# Autodesk Inventor assembly: Full Chassis - Full Assembly
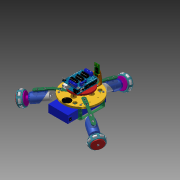
[picture p0: Inventor's stored thumbnail of the model, 180x180]
Saved by Autodesk Inventor 2014 (Build 180170000, 170)
## iProperties
Created: 2014-02-26
Part Number: Full Chassis - Full Assembly
Document SubType Name: Assembly
Designer: Spooner
Author: Spooner
## Documents named in this file (5)
- C:\Users\Spooner\Documents\Inventor\FerretBall Robot\3Pod\Inventor 2014 Files\Full Chassis - Full Assembly.iam
- C:\Users\Spooner\Documents\Inventor\FerretBall Robot\3Pod\Inventor 2014 Files\Main Body - Full Assembly.iam
- C:\Users\Spooner\Documents\Inventor\FerretBall Robot\3Pod\Inventor 2014 Files\Full Motor Arm (1 inch) with Kornylak Wheel.iam
- C:\Users\Spooner\Documents\Inventor\Content Center Files\R2014\en-US\JIS B 1111(1)\JIS B 1111 - M3x10(1).ipt
- C:\Users\Spooner\Documents\Inventor\Content Center Files\R2014\en-US\JIS B 1181 U\JIS B 1181 - B M3.ipt
## Components (16 placed, 4 different names)
1. Main Body - Full Assembly:1 [sub-assembly] — Insert:1, Mate:1, Insert:2, Mate:2, Insert:3, Mate:3, Insert:10, Insert:11, Insert:12, Insert:13, Insert:14, Insert:15
2. Full Motor Arm (1 inch) with Kornylak Wheel:1 [sub-assembly] — Insert:3, Mate:3, Insert:6, Insert:9, Angle:3, Angle:4
3. Full Motor Arm (1 inch) with Kornylak Wheel:2 [sub-assembly] — Insert:2, Mate:2, Insert:7, Insert:8, Angle:1, Angle:2
4. Full Motor Arm (1 inch) with Kornylak Wheel:3 [sub-assembly] — Insert:1, Mate:1, Insert:4, Insert:5, Angle:5, Angle:6
5. JIS B 1111 M3x10:1 — Insert:11
6. JIS B 1111 M3x10:2 — Insert:13
7. JIS B 1111 M3x10:3 — Insert:15
8. JIS B 1111 M3x10:4 — Insert:14
9. JIS B 1111 M3x10:5 — Insert:12
10. JIS B 1111 M3x10:6 — Insert:10
11. JIS B 1181 (unchamfered) - Metric B M3:1 — Insert:4, Angle:6
12. JIS B 1181 (unchamfered) - Metric B M3:2 — Insert:9, Angle:3
13. JIS B 1181 (unchamfered) - Metric B M3:3 — Insert:6, Angle:4
14. JIS B 1181 (unchamfered) - Metric B M3:4 — Insert:7, Angle:2
15. JIS B 1181 (unchamfered) - Metric B M3:5 — Insert:8, Angle:1
16. JIS B 1181 (unchamfered) - Metric B M3:6 — Insert:5, Angle:5
## Relationships (24: Insert 15, Angle 6, Mate 3)
- Insert:1: Main Body - Full Assembly:1 ↔ Full Motor Arm (1 inch) with Kornylak Wheel:3
- Mate:1: Main Body - Full Assembly:1 ↔ Full Motor Arm (1 inch) with Kornylak Wheel:3
- Insert:2: Main Body - Full Assembly:1 ↔ Full Motor Arm (1 inch) with Kornylak Wheel:2
- Mate:2: Main Body - Full Assembly:1 ↔ Full Motor Arm (1 inch) with Kornylak Wheel:2
- Insert:3: Main Body - Full Assembly:1 ↔ Full Motor Arm (1 inch) with Kornylak Wheel:1
- Mate:3: Main Body - Full Assembly:1 ↔ Full Motor Arm (1 inch) with Kornylak Wheel:1
- Insert:4: Full Motor Arm (1 inch) with Kornylak Wheel:3 ↔ JIS B 1181 (unchamfered) - Metric B M3:1
- Insert:5: Full Motor Arm (1 inch) with Kornylak Wheel:3 ↔ JIS B 1181 (unchamfered) - Metric B M3:6
- Insert:6: Full Motor Arm (1 inch) with Kornylak Wheel:1 ↔ JIS B 1181 (unchamfered) - Metric B M3:3
- Insert:7: Full Motor Arm (1 inch) with Kornylak Wheel:2 ↔ JIS B 1181 (unchamfered) - Metric B M3:4
- Insert:8: Full Motor Arm (1 inch) with Kornylak Wheel:2 ↔ JIS B 1181 (unchamfered) - Metric B M3:5
- Angle:1 (0 deg): Full Motor Arm (1 inch) with Kornylak Wheel:2 ↔ JIS B 1181 (unchamfered) - Metric B M3:5
- Angle:2 (0 deg): Full Motor Arm (1 inch) with Kornylak Wheel:2 ↔ JIS B 1181 (unchamfered) - Metric B M3:4
- Insert:9: Full Motor Arm (1 inch) with Kornylak Wheel:1 ↔ JIS B 1181 (unchamfered) - Metric B M3:2
- Angle:3 (0 deg): Full Motor Arm (1 inch) with Kornylak Wheel:1 ↔ JIS B 1181 (unchamfered) - Metric B M3:2
- Angle:4 (0 deg): Full Motor Arm (1 inch) with Kornylak Wheel:1 ↔ JIS B 1181 (unchamfered) - Metric B M3:3
- Angle:5 (0 deg): Full Motor Arm (1 inch) with Kornylak Wheel:3 ↔ JIS B 1181 (unchamfered) - Metric B M3:6
- Angle:6 (0 deg): Full Motor Arm (1 inch) with Kornylak Wheel:3 ↔ JIS B 1181 (unchamfered) - Metric B M3:1
- Insert:10: Main Body - Full Assembly:1 ↔ JIS B 1111 M3x10:6
- Insert:11: Main Body - Full Assembly:1 ↔ JIS B 1111 M3x10:1
- Insert:12: Main Body - Full Assembly:1 ↔ JIS B 1111 M3x10:5
- Insert:13: Main Body - Full Assembly:1 ↔ JIS B 1111 M3x10:2
- Insert:14: Main Body - Full Assembly:1 ↔ JIS B 1111 M3x10:4
- Insert:15: Main Body - Full Assembly:1 ↔ JIS B 1111 M3x10:3
